# Autodesk Inventor assembly: ExteriorBumperCar2
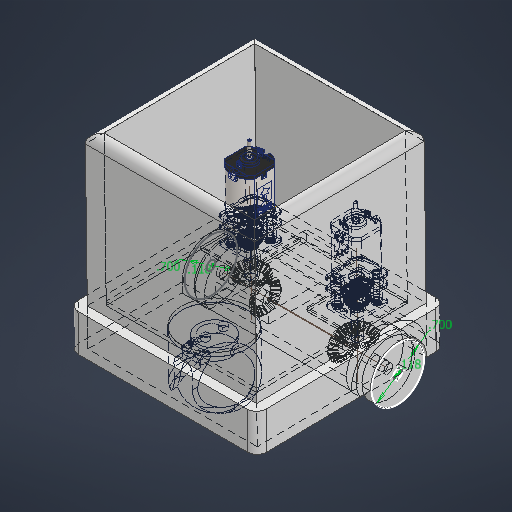
[picture p0: Inventor's stored thumbnail of the model, 512x512]
Saved by Autodesk Inventor 2026.1 (Build 301233000, 233)
## iProperties
Created: 2026-06-28
Part Number: ExteriorBumperCar2
Document SubType Name: Assembly
Designer: Kasi Pusuluri
Author: Kasi Pusuluri
## Documents named in this file (7)
- C:\Users\Kasi Pusuluri\Documents\Outpost 2026\BumperCarV2\ExteriorBumperCar2.iam
- C:\Users\Kasi Pusuluri\Documents\Outpost 2026\BumperCarV2\BumperBody.ipt
- C:\Users\Kasi Pusuluri\Documents\Outpost 2026\BumperCarV2\WheelAssembly.iam
- C:\Users\Kasi Pusuluri\Documents\Outpost 2026\BumperCarV2\BumperCaster2.ipt
- C:\Users\Kasi Pusuluri\Documents\Outpost 2026\BumperCarV2\Base.ipt
- C:\Users\Kasi Pusuluri\Documents\Outpost 2026\BumperCarV2\Battery2.ipt
- C:\Users\Kasi Pusuluri\Documents\Outpost 2026\BumperCarV2\WheelConnector.ipt
## Components (8 placed, 6 different names)
1. BumperBody:1 — Mate:3, Mate:4, Mate:5, Mate:6
2. WheelAssembly:1 [sub-assembly] — Mate:4, Mate:6
3. WheelAssembly:2 [sub-assembly] — Mate:3, Mate:5, Mate:7, Mate:8
4. BumperCaster2:1 — Rotational:9
5. Base:1 — Mate:7, Mate:8, Rotational:9
6. Battery2:1
7. WheelConnector:1
8. WheelConnector:2
## Relationships (7: Mate 6, RevoluteJoint 1)
- Mate:3: BumperBody:1 ↔ WheelAssembly:2
- Mate:4: BumperBody:1 ↔ WheelAssembly:1
- Mate:5: BumperBody:1 ↔ WheelAssembly:2
- Mate:6: BumperBody:1 ↔ WheelAssembly:1
- Mate:7: WheelAssembly:2 ↔ Base:1
- Mate:8: WheelAssembly:2 ↔ Base:1
- Rotational:9 [RevoluteJoint]: BumperCaster2:1 ↔ Base:1
